# Autodesk Inventor assembly: Assemb. Support AX12 pince
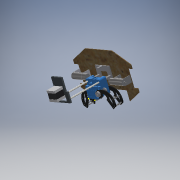
[picture p0: Inventor's stored thumbnail of the model, 180x180]
Saved by Autodesk Inventor 2017 (Build 210142000, 142)
## iProperties
Part Number: Assemb. Support AX12 pince
Material: Générique
Document SubType Name: Assembly
Designer: sasha
Author: sasha
## Documents named in this file (15)
- D:\Clemence\ENSEIRB\Eirbot\Pince\Final\Assemb. Support AX12 pince.iam
- D:\Clemence\ENSEIRB\Eirbot\Pince\Final\Support de 29mm de haut.ipt
- D:\Clemence\ENSEIRB\Eirbot\Pince\Final\Support AX12.ipt
- D:\Clemence\ENSEIRB\Eirbot\Pince\Final\Pince droite(2) .ipt
- D:\Clemence\ENSEIRB\Eirbot\Pince\Final\Pince gauche(2) .ipt
- D:\Clemence\ENSEIRB\Eirbot\Pince\Final\Tiges\tige 4,4.ipt
- D:\Clemence\ENSEIRB\Eirbot\Pince\tige 4,1.ipt
- D:\Clemence\ENSEIRB\Eirbot\Pince\Final\Tiges\Tube.ipt
- D:\Clemence\ENSEIRB\Eirbot\Pince\Final\Support haut.ipt
- D:\Clemence\ENSEIRB\Eirbot\Pince\Final\Moteur pas à pas.ipt
- D:\Clemence\ENSEIRB\Eirbot\Pince\Final\Support support AX12.ipt
- D:\Clemence\ENSEIRB\Eirbot\Base\base.ipt
- D:\Clemence\ENSEIRB\Eirbot\Base\Moteur.ipt
- D:\Clemence\ENSEIRB\Eirbot\Pince\Final\Support Poulie Bas.ipt
- D:\Clemence\ENSEIRB\Eirbot\Pince\Final\Tiges\3mm et 50 mm.ipt
## Components (26 placed, 14 different names)
1. Support de 29mm de haut:1 — Placage:1, Placage:2, Placage:3, Placage:6, Placage:7, Placage:8, Placage:9, Rotation:1, Cylindrique:1, Cylindrique:2, Placage:42, Placage:43
2. Support AX12:1 — Placage:1, Placage:2, Placage:3, Placage:44
3. Pince droite(2) :1 — Placage:17, Placage:18, Placage:20, Placage:21, Placage:35, Placage:36, Rotation:1
4. Pince gauche(2) :1 — Placage:8, Placage:9, Placage:13, Placage:14, Placage:22, Placage:23, Placage:24, Placage:25
5. Pince droite(2) :2 — Placage:16, Placage:19, Placage:30, Placage:31, Placage:32, Placage:33, Placage:34
6. Pince gauche(2) :2 — Placage:6, Placage:7, Placage:26, Placage:27, Placage:28, Placage:29
7. tige 4,4:1 — Placage:35, Placage:36
8. tige 4,4:2 — Placage:13, Placage:14
9. tige 4,1:1 — Placage:21, Placage:30
10. tige 4,1:2 — Placage:22, Placage:26
11. tige 4,1:3 — Placage:23, Placage:27
12. tige 4,1:4 — Placage:25, Placage:28
13. tige 4,1:5 — Placage:24, Placage:29
14. tige 4,1:6 — Placage:16, Placage:17, Placage:32
15. tige 4,1:7 — Placage:18, Placage:19, Placage:31, Placage:34
16. tige 4,1:8 — Placage:20, Placage:33
17. Tube:1 — Cylindrique:1, Placage:38, Placage:39, Placage:45, Placage:49, Placage:55
18. Tube:2 — Cylindrique:2, Placage:37, Placage:46, Placage:56
19. Support haut:1 — Placage:37, Placage:38, Placage:39, Placage:40, Placage:41
20. Moteur pas à pas:1 — Placage:40, Placage:41
21. Support support AX12:1 — Placage:42, Placage:43, Placage:44
22. base:1 — Placage:45, Placage:46, Placage:48, Placage:49, Placage:50, Placage:51, Placage:52, Placage:53, Placage:54
23. Moteur:1 — Placage:48, Placage:50
24. Moteur:2 — Placage:51, Placage:52, Placage:53
25. Support Poulie Bas:1 — Placage:54, Placage:55, Placage:56
26. 3mm et 50 mm:1
## Relationships (52: Mate 49, CylindricalJoint 2, RevoluteJoint 1)
- Placage:1 [Mate]: Support de 29mm de haut:1 ↔ Support AX12:1
- Placage:2 [Mate]: Support de 29mm de haut:1 ↔ Support AX12:1
- Placage:3 [Mate]: Support de 29mm de haut:1 ↔ Support AX12:1
- Placage:6 [Mate]: Support de 29mm de haut:1 ↔ Pince gauche(2) :2
- Placage:7 [Mate]: Support de 29mm de haut:1 ↔ Pince gauche(2) :2
- Placage:8 [Mate]: Support de 29mm de haut:1 ↔ Pince gauche(2) :1
- Placage:9 [Mate]: Support de 29mm de haut:1 ↔ Pince gauche(2) :1
- Placage:13 [Mate]: Pince gauche(2) :1 ↔ tige 4,4:2
- Placage:14 [Mate]: Pince gauche(2) :1 ↔ tige 4,4:2
- Placage:16 [Mate]: Pince droite(2) :2 ↔ tige 4,1:6
- Placage:17 [Mate]: Pince droite(2) :1 ↔ tige 4,1:6
- Placage:18 [Mate]: Pince droite(2) :1 ↔ tige 4,1:7
- Placage:19 [Mate]: Pince droite(2) :2 ↔ tige 4,1:7
- Placage:20 [Mate]: Pince droite(2) :1 ↔ tige 4,1:8
- Placage:21 [Mate]: Pince droite(2) :1 ↔ tige 4,1:1
- Placage:22 [Mate]: Pince gauche(2) :1 ↔ tige 4,1:2
- Placage:23 [Mate]: Pince gauche(2) :1 ↔ tige 4,1:3
- Placage:24 [Mate]: Pince gauche(2) :1 ↔ tige 4,1:5
- Placage:25 [Mate]: Pince gauche(2) :1 ↔ tige 4,1:4
- Placage:26 [Mate]: Pince gauche(2) :2 ↔ tige 4,1:2
- Placage:27 [Mate]: Pince gauche(2) :2 ↔ tige 4,1:3
- Placage:28 [Mate]: Pince gauche(2) :2 ↔ tige 4,1:4
- Placage:29 [Mate]: Pince gauche(2) :2 ↔ tige 4,1:5
- Placage:30 [Mate]: Pince droite(2) :2 ↔ tige 4,1:1
- Placage:31 [Mate]: Pince droite(2) :2 ↔ tige 4,1:7
- Placage:32 [Mate]: Pince droite(2) :2 ↔ tige 4,1:6
- Placage:33 [Mate]: Pince droite(2) :2 ↔ tige 4,1:8
- Placage:34 [Mate]: Pince droite(2) :2 ↔ tige 4,1:7
- Placage:35 [Mate]: Pince droite(2) :1 ↔ tige 4,4:1
- Placage:36 [Mate]: Pince droite(2) :1 ↔ tige 4,4:1
- Rotation:1 [RevoluteJoint]: Support de 29mm de haut:1 ↔ Pince droite(2) :1
- Cylindrique:1: Support de 29mm de haut:1 ↔ Tube:1
- Cylindrique:2: Support de 29mm de haut:1 ↔ Tube:2
- Placage:37 [Mate]: Tube:2 ↔ Support haut:1
- Placage:38 [Mate]: Tube:1 ↔ Support haut:1
- Placage:39 [Mate]: Tube:1 ↔ Support haut:1
- Placage:40 [Mate]: Support haut:1 ↔ Moteur pas à pas:1
- Placage:41 [Mate]: Support haut:1 ↔ Moteur pas à pas:1
- Placage:42 [Mate]: Support de 29mm de haut:1 ↔ Support support AX12:1
- Placage:43 [Mate]: Support de 29mm de haut:1 ↔ Support support AX12:1
- Placage:44 [Mate]: Support AX12:1 ↔ Support support AX12:1
- Placage:45 [Mate]: Tube:1 ↔ base:1
- Placage:46 [Mate]: Tube:2 ↔ base:1
- Placage:48 [Mate]: base:1 ↔ Moteur:1
- Placage:49 [Mate]: Tube:1 ↔ base:1
- Placage:50 [Mate]: base:1 ↔ Moteur:1
- Placage:51 [Mate]: base:1 ↔ Moteur:2
- Placage:52 [Mate]: base:1 ↔ Moteur:2
- Placage:53 [Mate]: base:1 ↔ Moteur:2
- Placage:54 [Mate]: base:1 ↔ Support Poulie Bas:1
- Placage:55 [Mate]: Tube:1 ↔ Support Poulie Bas:1
- Placage:56 [Mate]: Tube:2 ↔ Support Poulie Bas:1
